# Autodesk Inventor assembly: Rail_assy
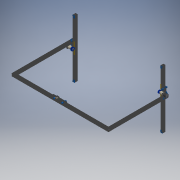
[picture p0: Inventor's stored thumbnail of the model, 180x180]
Saved by Autodesk Inventor 2019.4 (Build 234330000, 330)
## iProperties
Created: 2021-02-01
Part Number: Rail_assy
Document SubType Name: Assembly
Designer: Jorian Brusind
Author: Jorian Brusind
## Documents named in this file (4)
- C:\Users\Jorian Brusind\Documents\GitHub\PersonalProjects\HyperRail\Inventor Files\Rail_assy.iam
- C:\Users\Jorian Brusind\Documents\GitHub\PersonalProjects\HyperRail\Inventor Files\Rail_Assembly.iam
- C:\Users\Jorian Brusind\Documents\GitHub\PersonalProjects\Inventor Projects\Useful models\8020_Sets\IPT_40_Series\Extra_40_Series\HFS5-4060-4000\HFS5-4060-2125.ipt
- C:\Users\Jorian Brusind\Documents\GitHub\PersonalProjects\HyperRail\Inventor Files\YAxis_Carriage.iam
## Components (4 placed, 3 different names)
1. Rail_Assembly:1 [sub-assembly] — Mate:1, Flush:1, Flush:2, Flush:5, Mate:4
2. Rail_Assembly:2 [sub-assembly] — Flush:3, Mate:2, Flush:4, Flush:5, Mate:3
3. HFS5-4060-2125:1 — Mate:1, Flush:1, Flush:2, Flush:3, Mate:2, Flush:4, Mate:5, Mate:6
4. YAxis_Carriage:1 [sub-assembly] — Mate:5, Mate:6
## Relationships (11: Mate 6, Flush 5)
- Mate:1: Rail_Assembly:1 ↔ HFS5-4060-2125:1
- Flush:1: Rail_Assembly:1 ↔ HFS5-4060-2125:1
- Flush:2: Rail_Assembly:1 ↔ HFS5-4060-2125:1
- Flush:3: Rail_Assembly:2 ↔ HFS5-4060-2125:1
- Mate:2: Rail_Assembly:2 ↔ HFS5-4060-2125:1
- Flush:4: Rail_Assembly:2 ↔ HFS5-4060-2125:1
- Flush:5: Rail_Assembly:1 ↔ Rail_Assembly:2
- Mate:3: Rail_Assembly:2
- Mate:4: Rail_Assembly:1
- Mate:5: HFS5-4060-2125:1 ↔ YAxis_Carriage:1
- Mate:6 (7 mm): HFS5-4060-2125:1 ↔ YAxis_Carriage:1
